# Autodesk Inventor assembly: TempLoggerBox
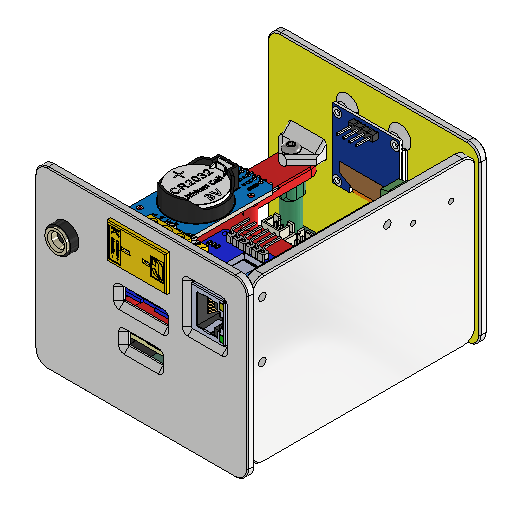
[picture p0: Inventor's stored thumbnail of the model, 512x512]
Saved by Autodesk Inventor 2026 (Build 300175050, 175E)
## iProperties
Created: 2025-07-16
Part Number: TempLoggerBox
Document SubType Name: Assembly
Designer: kuzmin
Author: kuzmin
## Documents named in this file (18)
- C:\Users\queezz\Dropbox\Drawings\PIHTI\ElectronicsBox\esp32-ambient-logger\TempLoggerBox.iam
- C:\Users\queezz\Dropbox\Drawings\PIHTI\ElectronicsBox\esp32-ambient-logger\TempLoggerRev1.iam
- C:\Users\queezz\Dropbox\Drawings\PIHTI\ElectronicsBox\esp32-ambient-logger\STEPs\ESP32-DevkitC32U.iam
- C:\Users\queezz\Dropbox\Drawings\PIHTI\ElectronicsBox\esp32-ambient-logger\temp-logger-base-plate.ipt
- C:\Users\queezz\Dropbox\Drawings\PIHTI\ElectronicsBox\esp32-ambient-logger\STEPs\w5500.iam
- C:\Users\queezz\Dropbox\Drawings\PIHTI\ElectronicsBox\esp32-ambient-logger\STEPs\DS3231 RTC\DS2321 RTC.ipt
- C:\Users\queezz\Dropbox\Drawings\PIHTI\ElectronicsBox\esp32-ambient-logger\STEPs\OLED-128x64-0.96.ipt
- C:\Users\queezz\Dropbox\Drawings\PIHTI\ElectronicsBox\esp32-ambient-logger\STEPs\Product_TF Micro SD Card Memory Modul .iam
- C:\Users\queezz\Dropbox\Drawings\PIHTI\ElectronicsBox\esp32-ambient-logger\temp-logger-side-plate.ipt
- C:\Users\queezz\Dropbox\Drawings\PIHTI\ElectronicsBox\esp32-ambient-logger\temp-logger-shelf.ipt
- C:\Users\queezz\Dropbox\Drawings\PIHTI\ElectronicsBox\esp32-ambient-logger\shaft-20mm.ipt
- C:\Users\queezz\Dropbox\Drawings\PIHTI\ElectronicsBox\TempController-v2\STEPs\Type-K Thermocouple Mini Socket\Type-K Thermocouple Mini Socket.iam
- C:\Users\queezz\Dropbox\Drawings\PIHTI\ContentCenter\Electrics\DC Jack Panel Mount Base.ipt
- C:\Users\queezz\Dropbox\Drawings\PIHTI\ElectronicsBox\esp32-ambient-logger\temp-logger-back-plate.ipt
- C:\Users\queezz\Dropbox\Drawings\PIHTI\ElectronicsBox\esp32-ambient-logger\STEPs\Adafruit_MAX31855.iam
- C:\Users\queezz\Dropbox\Drawings\PIHTI\ElectronicsBox\esp32-ambient-logger\temp-logger-front-plate.ipt
- C:\Users\queezz\Dropbox\Drawings\PIHTI\ContentCenter\Fastners\M3x6-BHCS.ipt
- C:\Users\queezz\Dropbox\Drawings\PIHTI\ContentCenter\Fastners\M3x8-BHCS.ipt
## Components (29 placed, 17 different names)
1. TempLoggerRev1:1 [sub-assembly] — Mate:1, Flush:1, Flush:2, Rigid:1, Rigid:3, Rigid:4, Rigid:5, Rigid:6
2. ESP32-DevkitC32U:1 [sub-assembly] — Mate:1, Flush:1, Flush:2
3. temp-logger-base-plate:1 — Rigid:1, Flush:7, Flush:8, Mate:8, Flush:11, Flush:12, Mate:15, Flush:14, Mate:16, Rotational:1, Rotational:2, Rigid:15, Rigid:16
4. w5500:1 [sub-assembly] — Rigid:7, Rigid:30
5. DS2321 RTC:1 — Rigid:25
6. OLED-128x64-0.96:1 — Rigid:10
7. Product_TF Micro SD Card Memory Modul :1 [sub-assembly] — Rigid:8
8. temp-logger-side-plate:1 — Flush:7, Flush:8, Rigid:7, Mate:12, Mate:13, Mate:14, Mate:18
9. temp-logger-shelf:1 — Mate:5, Mate:7, Rigid:8, Mate:18, Rigid:21, Rigid:22, Rigid:25
10. shaft-20mm:1 — Rigid:4
11. shaft-20mm:2 — Rigid:6
12. shaft-20mm:3 — Rigid:5
13. shaft-20mm:4 — Rigid:3, Mate:5, Mate:7
14. Type-K Thermocouple Mini Socket:1 [sub-assembly] — Mate:9, Mate:10, Mate:11
15. DC Jack Panel Mount Base:1 — Rigid:9
16. temp-logger-back-plate:1 — Mate:8, Mate:9, Mate:10, Mate:11, Rigid:9, Flush:13, Flush:14, Flush:16, Rigid:26, Rigid:29
17. Adafruit_MAX31855:1 [sub-assembly] — Mate:12, Mate:13, Mate:14
18. temp-logger-front-plate:1 — Mate:16, Flush:16, Rigid:10, Mate:19, Rigid:27, Rigid:28
19. Broached Hexagon Socket Button Head Cap Screw - Metric M3 x 0.5 x 6:11 — Rigid:30
20. BS 4168 : Part 6 Hexagon socket countersunk and button head screws - Metric series - Metric M3 x 8:1 — Rigid:29
21. BS 4168 : Part 6 Hexagon socket countersunk and button head screws - Metric series - Metric M3 x 8:2 — Rigid:28
22. BS 4168 : Part 6 Hexagon socket countersunk and button head screws - Metric series - Metric M3 x 8:3 — Rigid:27
23. BS 4168 : Part 6 Hexagon socket countersunk and button head screws - Metric series - Metric M3 x 8:4 — Rigid:26
24. Broached Hexagon Socket Button Head Cap Screw - Metric M3 x 0.5 x 6:9 — Rigid:22
25. Broached Hexagon Socket Button Head Cap Screw - Metric M3 x 0.5 x 6:10 — Rigid:21
26. Broached Hexagon Socket Button Head Cap Screw - Metric M3 x 0.5 x 6:5 — Rotational:1
27. Broached Hexagon Socket Button Head Cap Screw - Metric M3 x 0.5 x 6:6 — Rigid:15
28. Broached Hexagon Socket Button Head Cap Screw - Metric M3 x 0.5 x 6:7 — Rigid:16
29. Broached Hexagon Socket Button Head Cap Screw - Metric M3 x 0.5 x 6:8 — Rotational:2
## Relationships (44: WeldJoint 19, Mate 14, Flush 9, RevoluteJoint 2)
- Mate:1: TempLoggerRev1:1 ↔ ESP32-DevkitC32U:1
- Flush:1: TempLoggerRev1:1 ↔ ESP32-DevkitC32U:1
- Flush:2: TempLoggerRev1:1 ↔ ESP32-DevkitC32U:1
- Rigid:1 [WeldJoint]: TempLoggerRev1:1 ↔ temp-logger-base-plate:1
- Flush:7: temp-logger-base-plate:1 ↔ temp-logger-side-plate:1
- Rigid:3 [WeldJoint]: TempLoggerRev1:1 ↔ shaft-20mm:4
- Rigid:4 [WeldJoint]: TempLoggerRev1:1 ↔ shaft-20mm:1
- Rigid:5 [WeldJoint]: TempLoggerRev1:1 ↔ shaft-20mm:3
- Rigid:6 [WeldJoint]: TempLoggerRev1:1 ↔ shaft-20mm:2
- Flush:8: temp-logger-base-plate:1 ↔ temp-logger-side-plate:1
- Rigid:7 [WeldJoint]: w5500:1 ↔ temp-logger-side-plate:1
- Mate:5: temp-logger-shelf:1 ↔ shaft-20mm:4
- Mate:7: temp-logger-shelf:1 ↔ shaft-20mm:4
- Rigid:8 [WeldJoint]: Product_TF Micro SD Card Memory Modul :1 ↔ temp-logger-shelf:1
- Mate:8: temp-logger-base-plate:1 ↔ temp-logger-back-plate:1
- Mate:9: Type-K Thermocouple Mini Socket:1 ↔ temp-logger-back-plate:1
- Mate:10: Type-K Thermocouple Mini Socket:1 ↔ temp-logger-back-plate:1
- Mate:11: Type-K Thermocouple Mini Socket:1 ↔ temp-logger-back-plate:1
- Rigid:9 [WeldJoint]: DC Jack Panel Mount Base:1 ↔ temp-logger-back-plate:1
- Mate:12: temp-logger-side-plate:1 ↔ Adafruit_MAX31855:1
- Mate:13: temp-logger-side-plate:1 ↔ Adafruit_MAX31855:1
- Mate:14: temp-logger-side-plate:1 ↔ Adafruit_MAX31855:1
- Flush:11: temp-logger-base-plate:1
- Flush:12: temp-logger-base-plate:1
- Mate:15: temp-logger-base-plate:1
- Flush:13: temp-logger-back-plate:1
- Flush:14 (3 mm): temp-logger-base-plate:1 ↔ temp-logger-back-plate:1
- Mate:16: temp-logger-base-plate:1 ↔ temp-logger-front-plate:1
- Flush:16: temp-logger-back-plate:1 ↔ temp-logger-front-plate:1
- Rigid:10 [WeldJoint]: OLED-128x64-0.96:1 ↔ temp-logger-front-plate:1
- Rotational:1 [RevoluteJoint]: temp-logger-base-plate:1 ↔ Broached Hexagon Socket Button Head Cap Screw - Metric M3 x 0.5 x 6:5
- Rotational:2 [RevoluteJoint]: temp-logger-base-plate:1 ↔ Broached Hexagon Socket Button Head Cap Screw - Metric M3 x 0.5 x 6:8
- Rigid:15 [WeldJoint]: temp-logger-base-plate:1 ↔ Broached Hexagon Socket Button Head Cap Screw - Metric M3 x 0.5 x 6:6
- Rigid:16 [WeldJoint]: temp-logger-base-plate:1 ↔ Broached Hexagon Socket Button Head Cap Screw - Metric M3 x 0.5 x 6:7
- Mate:18 (4.5 mm): temp-logger-side-plate:1 ↔ temp-logger-shelf:1
- Rigid:21 [WeldJoint]: temp-logger-shelf:1 ↔ Broached Hexagon Socket Button Head Cap Screw - Metric M3 x 0.5 x 6:10
- Rigid:22 [WeldJoint]: temp-logger-shelf:1 ↔ Broached Hexagon Socket Button Head Cap Screw - Metric M3 x 0.5 x 6:9
- Rigid:25 [WeldJoint]: DS2321 RTC:1 ↔ temp-logger-shelf:1
- Mate:19: temp-logger-front-plate:1
- Rigid:26 [WeldJoint]: temp-logger-back-plate:1 ↔ BS 4168 : Part 6 Hexagon socket countersunk and button head screws - Metric series - Metric M3 x 8:4
- Rigid:27 [WeldJoint]: temp-logger-front-plate:1 ↔ BS 4168 : Part 6 Hexagon socket countersunk and button head screws - Metric series - Metric M3 x 8:3
- Rigid:28 [WeldJoint]: temp-logger-front-plate:1 ↔ BS 4168 : Part 6 Hexagon socket countersunk and button head screws - Metric series - Metric M3 x 8:2
- Rigid:29 [WeldJoint]: temp-logger-back-plate:1 ↔ BS 4168 : Part 6 Hexagon socket countersunk and button head screws - Metric series - Metric M3 x 8:1
- Rigid:30 [WeldJoint]: w5500:1 ↔ Broached Hexagon Socket Button Head Cap Screw - Metric M3 x 0.5 x 6:11
